# Autodesk Inventor assembly: Landing_leg_simulator.ipt
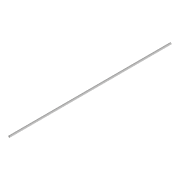
[picture p0: Inventor's stored thumbnail of the model, 180x180]
Saved by Autodesk Inventor 2022 (Build 260153000, 153)
## iProperties
Created: 2022-04-29
Part Number: Landing_leg_simulator.ipt
Document SubType Name: Assembly
Designer: dell
Author: dell
## Documents named in this file (2)
- D:\xxxx\Uni\Part IV\MECHENG_700\Part_IV_project_CAD\Bird_skeleton_prototypes\Wing_drone_V1\Landing_leg_simulator.ipt.iam
- D:\xxxx\Uni\Part IV\MECHENG_700\Part_IV_project_CAD\Bird_skeleton_prototypes\Wing_drone_V1\Landing_leg_rod_simulator.ipt
## Components (3 placed, 1 different names)
1. Landing_leg_rod_simulator:1 — Mate:1, Mate:2
2. Landing_leg_rod_simulator:2 — Mate:1, Mate:2, Mate:3, Mate:4
3. Landing_leg_rod_simulator:3 — Mate:3, Mate:4
## Relationships (4: Mate 4)
- Mate:1: Landing_leg_rod_simulator:1 ↔ Landing_leg_rod_simulator:2
- Mate:2: Landing_leg_rod_simulator:1 ↔ Landing_leg_rod_simulator:2
- Mate:3: Landing_leg_rod_simulator:2 ↔ Landing_leg_rod_simulator:3
- Mate:4: Landing_leg_rod_simulator:2 ↔ Landing_leg_rod_simulator:3
